# Autodesk Inventor assembly: extruder
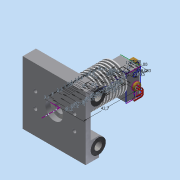
[picture p0: Inventor's stored thumbnail of the model, 180x180]
Saved by Autodesk Inventor 2015 (Build 190159000, 159)
## iProperties
Created: 2016-09-08
Part Number: extruder
Document SubType Name: Assembly
Designer: Dustin
Author: Dustin
## Documents named in this file (4)
- E:\Documents\3D Printer\LetzteBot3DPrinter\Inventor Files\IAM Files\extruder.iam
- E:\Documents\3D Printer\LetzteBot3DPrinter\Inventor Files\E3D-HotEnd\E3D-HotEnd.iam
- E:\Documents\3D Printer\LetzteBot3DPrinter\Inventor Files\IPT Files\Small Parts\Extruder mount.ipt
- E:\Documents\3D Printer\LetzteBot3DPrinter\Inventor Files\IPT Files\LM6UU.ipt
## Components (6 placed, 3 different names)
1. E3D-HotEnd:1 [sub-assembly] — Tangent:1, Insert:1
2. Extruder mount:1 — Tangent:1, Insert:1, Tangent:2, Flush:1, Tangent:3, Flush:2, Tangent:4, Flush:3, Tangent:5, Flush:4
3. LM6UU:1 — Tangent:3, Flush:2
4. LM6UU:2 — Tangent:2, Flush:1
5. LM6UU:3 — Tangent:4, Flush:3
6. LM6UU:4 — Tangent:5, Flush:4
## Relationships (10: Tangent 5, Flush 4, Insert 1)
- Tangent:1: E3D-HotEnd:1 ↔ Extruder mount:1
- Insert:1: E3D-HotEnd:1 ↔ Extruder mount:1
- Tangent:2: Extruder mount:1 ↔ LM6UU:2
- Flush:1: Extruder mount:1 ↔ LM6UU:2
- Tangent:3: Extruder mount:1 ↔ LM6UU:1
- Flush:2: Extruder mount:1 ↔ LM6UU:1
- Tangent:4: Extruder mount:1 ↔ LM6UU:3
- Flush:3: Extruder mount:1 ↔ LM6UU:3
- Tangent:5: Extruder mount:1 ↔ LM6UU:4
- Flush:4: Extruder mount:1 ↔ LM6UU:4
